# Autodesk Inventor assembly: Assy_fork_connection
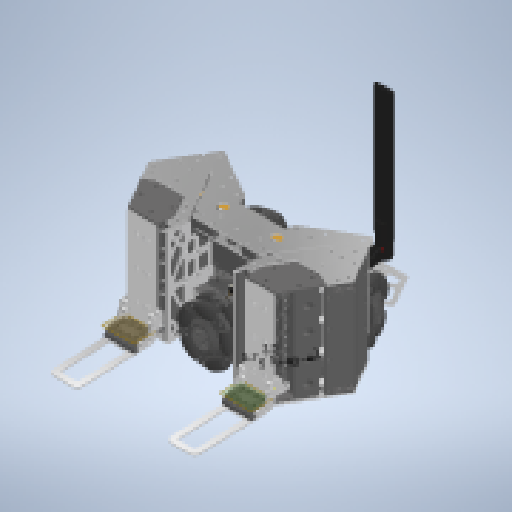
[picture p0: Inventor's stored thumbnail of the model, 512x512]
Saved by Autodesk Inventor 2024.1 (Build 281209000, 209)
## iProperties
Created: 2025-03-04
Part Number: Assy_fork_connection
Document SubType Name: Assembly
Designer: hibik
Author: hibik
## Documents named in this file (9)
- C:\Users\hibik\Documents\Robomech\RESCUE\ORCA\hard\Assy_fork_connection.iam
- C:\Users\hibik\Documents\Robomech\RESCUE\ORCA\hard\Assy_foot.iam
- C:\Users\hibik\Documents\Robomech\RESCUE\ORCA\hard\flame_base\base2fork_connecter_front.ipt
- C:\Users\hibik\Documents\Robomech\RESCUE\ORCA\hard\flame_base\base2fork_connecter_back.ipt
- C:\Users\hibik\Documents\Robomech\RESCUE\ORCA\hard\fork\Assy_upper_plate.iam
- C:\Users\hibik\Documents\Robomech\RESCUE\ORCA\hard\fork\belt.ipt
- C:\Users\hibik\Documents\Robomech\RESCUE\ORCA\hard\fork\right\Assy_fork_right.iam
- C:\Users\hibik\Documents\Robomech\RESCUE\ORCA\hard\fork\left\Assy_fork_left.iam
- C:\Users\hibik\Documents\Robomech\RESCUE\ORCA\hard\board\CORE_model\md.iam
## Components (10 placed, 8 different names)
1. Assy_foot:1 [sub-assembly] — 挿入:1, 挿入:2, 挿入:3, 挿入:4, 挿入:12, 挿入:15, 挿入:16, 挿入:17, 挿入:18, メイト:2, 挿入:23, 角度:1
2. base2fork_connecter_back:1 — 挿入:1, 挿入:2, 挿入:20
3. base2fork_connecter_front:1 — 挿入:3, 挿入:4, 挿入:19
4. Assy_upper_plate:1 [sub-assembly] — 挿入:12, フラッシュ:1, メイト:1
5. belt:1 — フラッシュ:1, メイト:1
6. Assy_fork_right:1 [sub-assembly] — 挿入:19, 挿入:20
7. base2fork_connecter_back:2 — 挿入:17, 挿入:18, 挿入:22
8. base2fork_connecter_front:2 — 挿入:15, 挿入:16, 挿入:21
9. Assy_fork_left:1 [sub-assembly] — 挿入:21, 挿入:22
10. md:1 [sub-assembly] — メイト:2, 挿入:23, 角度:1
## Relationships (18: Insert 14, Mate 2, Flush 1, Angle 1)
- 挿入:1 [Insert]: Assy_foot:1 ↔ base2fork_connecter_back:1
- 挿入:2 [Insert]: Assy_foot:1 ↔ base2fork_connecter_back:1
- 挿入:3 [Insert]: Assy_foot:1 ↔ base2fork_connecter_front:1
- 挿入:4 [Insert]: Assy_foot:1 ↔ base2fork_connecter_front:1
- 挿入:12 [Insert]: Assy_foot:1 ↔ Assy_upper_plate:1
- フラッシュ:1 [Flush]: Assy_upper_plate:1 ↔ belt:1
- メイト:1 [Mate] (1 mm): Assy_upper_plate:1 ↔ belt:1
- 挿入:15 [Insert]: Assy_foot:1 ↔ base2fork_connecter_front:2
- 挿入:16 [Insert]: Assy_foot:1 ↔ base2fork_connecter_front:2
- 挿入:17 [Insert]: Assy_foot:1 ↔ base2fork_connecter_back:2
- 挿入:18 [Insert]: Assy_foot:1 ↔ base2fork_connecter_back:2
- 挿入:19 [Insert]: base2fork_connecter_front:1 ↔ Assy_fork_right:1
- 挿入:20 [Insert]: base2fork_connecter_back:1 ↔ Assy_fork_right:1
- 挿入:21 [Insert]: base2fork_connecter_front:2 ↔ Assy_fork_left:1
- 挿入:22 [Insert]: base2fork_connecter_back:2 ↔ Assy_fork_left:1
- メイト:2 [Mate]: Assy_foot:1 ↔ md:1
- 挿入:23 [Insert]: Assy_foot:1 ↔ md:1
- 角度:1 [Angle] (0 deg): Assy_foot:1 ↔ md:1
